# Autodesk Inventor assembly: Cockpit_battery_back_door
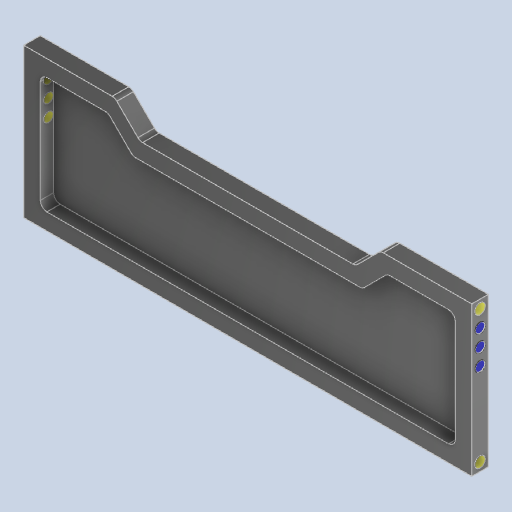
[picture p0: Inventor's stored thumbnail of the model, 512x512]
Saved by Autodesk Inventor 2022.3 (Build 263350000, 350)
## iProperties
Created: 2023-05-18
Part Number: Cockpit_battery_back_door
Document SubType Name: Assembly
Designer: Masato Kubotera
Author: Masato Kubotera
## Documents named in this file (3)
- C:\Users\Masato\Desktop\SUSTAINA-OP\UpperBody\Cockpit\Cockpit_battery_back_door.iam
- C:\Users\Masato\Desktop\SUSTAINA-OP\UpperBody\Cockpit\Cockpit_battery_back_door.ipt
- C:\Users\Masato\Desktop\SUSTAINA-OP\ReadyMade\Neodymium_magnet_Phi3_T3.ipt
## Components (7 placed, 2 different names)
1. Cockpit_battery_back_door:1 — Flush:1, Flush:2, Flush:3, Insert:1, Insert:2, Insert:3, Insert:4, Insert:5, Insert:6
2. Neodymium_magnet_Phi3_T3:1 — Insert:1
3. Neodymium_magnet_Phi3_T3:2 — Insert:2
4. Neodymium_magnet_Phi3_T3:3 — Insert:3
5. Neodymium_magnet_Phi3_T3:4 — Insert:4
6. Neodymium_magnet_Phi3_T3:5 — Insert:5
7. Neodymium_magnet_Phi3_T3:6 — Insert:6
## Relationships (9: Insert 6, Flush 3)
- Flush:1: Cockpit_battery_back_door:1
- Flush:2: Cockpit_battery_back_door:1
- Flush:3: Cockpit_battery_back_door:1
- Insert:1: Cockpit_battery_back_door:1 ↔ Neodymium_magnet_Phi3_T3:1
- Insert:2: Cockpit_battery_back_door:1 ↔ Neodymium_magnet_Phi3_T3:2
- Insert:3: Cockpit_battery_back_door:1 ↔ Neodymium_magnet_Phi3_T3:3
- Insert:4: Cockpit_battery_back_door:1 ↔ Neodymium_magnet_Phi3_T3:4
- Insert:5: Cockpit_battery_back_door:1 ↔ Neodymium_magnet_Phi3_T3:5
- Insert:6: Cockpit_battery_back_door:1 ↔ Neodymium_magnet_Phi3_T3:6
